# Autodesk Inventor assembly: arm_des_1
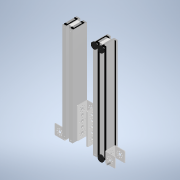
[picture p0: Inventor's stored thumbnail of the model, 180x180]
Saved by Autodesk Inventor 2020.1 (Build 241239000, 239)
## iProperties
Created: 2019-12-04
Part Number: arm_des_1
Document SubType Name: Assembly
Designer: tbloo
Author: tbloo
## Documents named in this file (9)
- C:\Users\tbloo\Documents\GitHub\AO_Robotics\CAD\Projects\Timothy Bloot\arm_des_1.iam
- C:\Users\tbloo\Documents\GitHub\AO_Robotics\CAD\Projects\Timothy Bloot\12in_Slide\12in-slide-pt_1.ipt
- C:\Users\tbloo\Documents\GitHub\AO_Robotics\CAD\Projects\Timothy Bloot\12in_Slide\12in-slide-pt_2.ipt
- C:\Users\tbloo\Documents\GitHub\AO_Robotics\CAD\Projects\Timothy Bloot\12in_Slide\12in-slide-pt_3.ipt
- C:\Users\tbloo\Documents\GitHub\AO_Robotics\CAD\Projects\Timothy Bloot\AM_Pulley.ipt
- C:\Users\tbloo\Documents\GitHub\AO_Robotics\CAD\Parts Kits\FTC Tetrix KOP Organized (7-24-19)\Frame Hardware\Tetrix_39065.ipt
- C:\Users\tbloo\Documents\GitHub\AO_Robotics\CAD\Parts Kits\FTC Tetrix KOP Organized (7-24-19)\Nuts and Bolts\Tetrix_39097.ipt
- C:\Users\tbloo\Documents\GitHub\AO_Robotics\CAD\Projects\Timothy Bloot\slide spacer.ipt
- C:\Users\tbloo\Documents\GitHub\AO_Robotics\CAD\Parts Kits\FTC Tetrix KOP Organized (7-24-19)\Frame Hardware\Tetrix_39066.ipt
## Components (25 placed, 8 different names)
1. 12in-slide-pt_1:1 — Slider:1, Rotational:1, Flush:11, Flush:12, Mate:6
2. 12in-slide-pt_2:1 — Slider:1, Slider:2
3. 12in-slide-pt_3:1 — Slider:2, Mate:2, Flush:3, Flush:4, Mate:3, Flush:5, Flush:6
4. 12in-slide-pt_1:2 — Slider:3, Rotational:2, Rotational:3, Mate:4, Flush:7
5. 12in-slide-pt_2:2 — Slider:3, Flush:2
6. 12in-slide-pt_3:2 — Flush:1, Mate:1, Flush:8
7. AM_Pulley:1 — Rotational:1
8. AM_Pulley:2 — Rotational:2
9. AM_Pulley:3 — Rotational:3
10. Tetrix_39065:1 — Flush:1, Mate:1, Flush:2, Rigid:1
11. Tetrix_39097:1 — Rigid:1
12. slide spacer:1 — Mate:2, Flush:3, Flush:4
13. slide spacer:2 — Mate:3, Flush:5, Flush:6, Mate:4, Flush:7, Flush:8
14. Tetrix_39066:1 — Mate:5, Flush:9, Flush:10, Mate:11, Flush:21, Flush:22
15. Tetrix_39066:2 — Mate:5, Flush:9, Flush:10, Flush:11, Flush:12, Mate:6
16. 12in-slide-pt_1:3 — Mate:11, Flush:21, Flush:22
17. 12in-slide-pt_2:3
18. 12in-slide-pt_3:3
19. 12in-slide-pt_1:4
20. 12in-slide-pt_2:4
21. 12in-slide-pt_3:4
22. Tetrix_39065:2
23. Tetrix_39097:2
24. slide spacer:3
25. slide spacer:4
## Relationships (46: Flush 22, Mate 11, TranslationJoint 8, RevoluteJoint 3, WeldJoint 2)
- Slider:1 [TranslationJoint]: 12in-slide-pt_1:1 ↔ 12in-slide-pt_2:1
- Slider:2 [TranslationJoint]: 12in-slide-pt_2:1 ↔ 12in-slide-pt_3:1
- Slider:3 [TranslationJoint]: 12in-slide-pt_1:2 ↔ 12in-slide-pt_2:2
- [TranslationJoint]: 12in-slide-pt_2:2 ↔ 12in-slide-pt_3:2
- Rotational:1 [RevoluteJoint]: 12in-slide-pt_1:1 ↔ AM_Pulley:1
- Rotational:2 [RevoluteJoint]: 12in-slide-pt_1:2 ↔ AM_Pulley:2
- Rotational:3 [RevoluteJoint]: 12in-slide-pt_1:2 ↔ AM_Pulley:3
- Flush:1 (-12.7 mm): 12in-slide-pt_3:2 ↔ Tetrix_39065:1
- Mate:1: 12in-slide-pt_3:2 ↔ Tetrix_39065:1
- Flush:2: 12in-slide-pt_2:2 ↔ Tetrix_39065:1
- Rigid:1 [WeldJoint]: Tetrix_39065:1 ↔ Tetrix_39097:1
- Mate:2: 12in-slide-pt_3:1 ↔ slide spacer:1
- Flush:3: 12in-slide-pt_3:1 ↔ slide spacer:1
- Flush:4: 12in-slide-pt_3:1 ↔ slide spacer:1
- Mate:3: 12in-slide-pt_3:1 ↔ slide spacer:2
- Flush:5: 12in-slide-pt_3:1 ↔ slide spacer:2
- Flush:6: 12in-slide-pt_3:1 ↔ slide spacer:2
- Mate:4: 12in-slide-pt_1:2 ↔ slide spacer:2
- Flush:7: 12in-slide-pt_1:2 ↔ slide spacer:2
- Flush:8: 12in-slide-pt_3:2 ↔ slide spacer:2
- Mate:5: Tetrix_39066:1 ↔ Tetrix_39066:2
- Flush:9: Tetrix_39066:1 ↔ Tetrix_39066:2
- Flush:10: Tetrix_39066:1 ↔ Tetrix_39066:2
- Flush:11: 12in-slide-pt_1:1 ↔ Tetrix_39066:2
- Flush:12: 12in-slide-pt_1:1 ↔ Tetrix_39066:2
- Mate:6: 12in-slide-pt_1:1 ↔ Tetrix_39066:2
- [TranslationJoint]: 12in-slide-pt_1:3 ↔ 12in-slide-pt_2:3
- [TranslationJoint]: 12in-slide-pt_2:3 ↔ 12in-slide-pt_3:3
- [TranslationJoint]: 12in-slide-pt_1:4 ↔ 12in-slide-pt_2:4
- [TranslationJoint]: 12in-slide-pt_2:4 ↔ 12in-slide-pt_3:4
- [Flush] (-12.7 mm): 12in-slide-pt_3:4 ↔ Tetrix_39065:2
- [Mate]: 12in-slide-pt_3:4 ↔ Tetrix_39065:2
- [Flush]: 12in-slide-pt_2:4 ↔ Tetrix_39065:2
- [WeldJoint]: Tetrix_39065:2 ↔ Tetrix_39097:2
- [Mate]: 12in-slide-pt_3:3 ↔ slide spacer:3
- [Flush]: 12in-slide-pt_3:3 ↔ slide spacer:3
- [Flush]: 12in-slide-pt_3:3 ↔ slide spacer:3
- [Mate]: 12in-slide-pt_3:3 ↔ slide spacer:4
- [Flush]: 12in-slide-pt_3:3 ↔ slide spacer:4
- [Flush]: 12in-slide-pt_3:3 ↔ slide spacer:4
- [Mate]: 12in-slide-pt_1:4 ↔ slide spacer:4
- [Flush]: 12in-slide-pt_1:4 ↔ slide spacer:4
- [Flush]: 12in-slide-pt_3:4 ↔ slide spacer:4
- Mate:11: Tetrix_39066:1 ↔ 12in-slide-pt_1:3
- Flush:21: Tetrix_39066:1 ↔ 12in-slide-pt_1:3
- Flush:22: Tetrix_39066:1 ↔ 12in-slide-pt_1:3
## Named parameters: d8_d0 = 0 mm, d9_d1 = 0 mm, d10_d2 = 0 mm, d11_d3 = -152.4 mm, d12_d4 = 0 mm, d13_d5 = 0 mm, d14_d6 = -5.73691 mm, d15_d7 = -152.4 mm, d41_d26 = 0 mm, d42_d27 = 0 mm, d43_d28 = 0 mm, d44_d29 = 0 mm, d45_d30 = 0 mm, d46_d31 = 0 mm, d47_d32 = 0 mm, d48_d33 = 0 mm, d49_d34 = 0 mm, d50_d8_d0 = 0 mm, d51_d9_d1 = 0 mm, d52_d10_d2 = 0 mm, d53_d11_d3 = -152.4 mm, d54_d12_d4 = 0 mm, d55_d13_d5 = 0 mm, d56_d14_d6 = 0 mm, d57_d15_d7 = -152.4 mm, d64_d22 = -12.7 mm, d65_d23 = 0 mm, d66_d24 = 0 mm, d67_d25 = 0 mm, d68_d0 = 0 mm, d69_d1 = 0 mm, d70_d2 = 0 mm, d71_d3 = -152.4 mm, d72_d4 = 0 mm, d73_d5 = 0 mm, d74_d6 = 0 mm, d75_d7 = -152.4 mm
